# Autodesk Inventor assembly: Conjunto_para_piezas
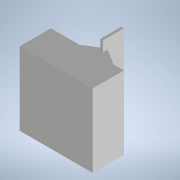
[picture p0: Inventor's stored thumbnail of the model, 180x180]
Saved by Autodesk Inventor 2021 (Build 250183000, 183)
## iProperties
Created: 2022-01-26
Part Number: Conjunto_para_piezas
Document SubType Name: Assembly
Designer: pc
Author: pc
## Documents named in this file (3)
- D:\pc\Documentos\Semestres\2021-2\ROBOTICA\proyectofinal\CADS\Conjunto_para_piezas.iam
- D:\pc\Documentos\Semestres\2021-2\ROBOTICA\proyectofinal\CADS\Base_rotativa.ipt
- D:\pc\Documentos\Semestres\2021-2\ROBOTICA\proyectofinal\CADS\Soporte.ipt
## Components (2 placed, 2 different names)
1. Base_rotativa:1 — Ángulo:1, Coincidencia:1, Coincidencia:2
2. Soporte:1 — Ángulo:1, Coincidencia:1, Coincidencia:2
## Relationships (3: Mate 2, Angle 1)
- Ángulo:1 [Angle] (0 deg): Base_rotativa:1 ↔ Soporte:1
- Coincidencia:1 [Mate]: Base_rotativa:1 ↔ Soporte:1
- Coincidencia:2 [Mate]: Base_rotativa:1 ↔ Soporte:1
